# Autodesk Inventor assembly: MotorAssembly
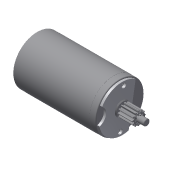
[picture p0: Inventor's stored thumbnail of the model, 180x180]
Saved by Autodesk Inventor 2013 SP1 (Build 170176100, 176)
## iProperties
Created: 2013-12-03
Part Number: MotorAssembly
Document SubType Name: Assembly
Designer: robotics
Author: robotics
## Documents named in this file (6)
- C:\Users\robotics\Documents\GitHub\2014-Preseason-Single-Speed-Gearbox\manufacture\assemblies\LeftMotorAssembly.iam
- C:\Users\robotics\Documents\GitHub\2014-Preseason-Single-Speed-Gearbox\buy\VexPro\Gears\217-2614-Rev02-STEP\Imported Components\217-2614-002\217-2614-002.ipt
- C:\Users\robotics\Documents\GitHub\2014-Preseason-Single-Speed-Gearbox\buy\VexPro\Gears\217-2614-Rev02-STEP\Imported Components\217-2614-001\217-2614-001.ipt
- C:\Users\robotics\Documents\GitHub\2014-Preseason-Single-Speed-Gearbox\buy\VexPro\Gears\217-2614-Rev02-STEP\Imported Components\217-2761-001 rev1\217-2761-001 rev1.ipt
- C:\Users\robotics\Documents\GitHub\2014-Preseason-Single-Speed-Gearbox\buy\VexPro\Motors\217-2000-STEP\Imported Components\217-2000\217-2000.ipt
- C:\Users\robotics\Documents\GitHub\2014-Preseason-Single-Speed-Gearbox\manufacture\acrylic\MotorSpacer.ipt
## Components (5 placed, 5 different names)
1. 217-2000:1 — Mate:1, Mate:2, Mate:3, Mate:4, Mate:5, Mate:7, Mate:8, Mate:9, Mate:10
2. 217-2614-002:1 — Mate:5, Mate:6
3. 217-2614-001:1 — Mate:4, Mate:6, Mate:7
4. 217-2761-001 rev1:1 — Mate:1, Mate:2, Mate:3
5. MotorSpacer:1 — Mate:8, Mate:9, Mate:10
## Relationships (10: Mate 10)
- Mate:1: 217-2000:1 ↔ 217-2761-001 rev1:1
- Mate:2: 217-2000:1 ↔ 217-2761-001 rev1:1
- Mate:3: 217-2000:1 ↔ 217-2761-001 rev1:1
- Mate:4: 217-2000:1 ↔ 217-2614-001:1
- Mate:5: 217-2000:1 ↔ 217-2614-002:1
- Mate:6: 217-2614-002:1 ↔ 217-2614-001:1
- Mate:7 (2 mm): 217-2000:1 ↔ 217-2614-001:1
- Mate:8: 217-2000:1 ↔ MotorSpacer:1
- Mate:9: 217-2000:1 ↔ MotorSpacer:1
- Mate:10: 217-2000:1 ↔ MotorSpacer:1
